# Autodesk Inventor assembly: R2_上昇機構
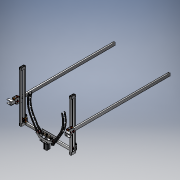
[picture p0: Inventor's stored thumbnail of the model, 180x180]
Saved by Autodesk Inventor 2019.4 (Build 234330000, 330)
## iProperties
Created: 2021-12-04
Part Number: R2_上昇機構
Material: 一般
Document SubType Name: Assembly
Designer: 堀川皓史
Mass: 2467.94 g
Surface Area: 9954.17 cm^2
Volume: 1031.77 cm^3
Density: 2.39196 g/cm^3
Author: 堀川皓史
## Documents named in this file (17)
- C:\Users\堀川皓史\Desktop\ロボ研\NHKフォルダ\2022NHKロボコン\R2_version1\R2_上昇機構.iam
- C:\Users\堀川皓史\Desktop\ロボ研\NHKフォルダ\2022NHKロボコン\R2_version1\上昇機構_内側板.ipt
- C:\Users\堀川皓史\Desktop\ロボ研\NHKフォルダ\2022NHKロボコン\R2_version1\上昇機構_外側板.ipt
- C:\Users\堀川皓史\Desktop\ロボ研\NHKフォルダ\2022NHKロボコン\R2_version1\上昇機構_固定軸ベアリングの.ipt
- C:\Users\堀川皓史\Desktop\ロボ研\NHKフォルダ\2022NHKロボコン\R2_version1\ベアリング_6-19-6.ipt
- C:\Users\堀川皓史\Desktop\ロボ研\NHKフォルダ\2022NHKロボコン\R2_version1\上昇機構_角柱1.ipt
- C:\Users\堀川皓史\Desktop\ロボ研\NHKフォルダ\2022NHKロボコン\R2_version1\上昇機構_固定具1.ipt
- C:\Users\堀川皓史\Desktop\ロボ研\NHKフォルダ\2022NHKロボコン\R2_version1\スペーサ_6.1-7_3Dプリンタ.ipt
- C:\Users\堀川皓史\Desktop\ロボ研\NHKフォルダ\2022NHKロボコン\R2_version1\軸_6-24.ipt
- C:\Users\堀川皓史\Desktop\ロボ研\NHKフォルダ\2022NHKロボコン\R2_version1\上昇機構_角柱3.ipt
- C:\Users\堀川皓史\Desktop\ロボ研\NHKフォルダ\2022NHKロボコン\R2_version1\上昇機構_角柱4.ipt
- C:\Users\堀川皓史\Desktop\ロボ研\NHKフォルダ\2022NHKロボコン\R2_version1\上昇機構_側板1.ipt
- C:\Users\堀川皓史\Desktop\ロボ研\NHKフォルダ\2022NHKロボコン\R2_version1\前後機構_上側板.ipt
- C:\Users\堀川皓史\Desktop\ロボ研\NHKフォルダ\2022NHKロボコン\R2_version1\前後機構_下側板.ipt
- C:\Users\堀川皓史\Desktop\ロボ研\NHKフォルダ\2022NHKロボコン\R2_version1\軸_3.2-8_特殊.ipt
- C:\Users\堀川皓史\Desktop\ロボ研\NHKフォルダ\2022NHKロボコン\R2_version1\ベアリング_3-7-3.ipt
- C:\Users\堀川皓史\Desktop\ロボ研\NHKフォルダ\2022NHKロボコン\R2_version1\R2_ハンド.iam
## Components (97 placed, 16 different names)
1. 上昇機構_内側板:1 — 挿入:57, 挿入:58, メイト:17, 挿入:63, 挿入:66, 挿入:67, 挿入:81, 挿入:82
2. 上昇機構_外側板:1 — 挿入:59, 挿入:60, 挿入:61, 挿入:62, メイト:20, メイト:21, 挿入:72, 挿入:73
3. 上昇機構_固定軸ベアリングの:1 — 挿入:61, 挿入:62, メイト:19
4. 上昇機構_固定軸ベアリングの:2 — 挿入:59, 挿入:60, メイト:18
5. 上昇機構_固定軸ベアリングの:3 — 挿入:57, 挿入:58, メイト:16
6. ベアリング_6-19-6:1 — メイト:16, メイト:17, 正接:4
7. ベアリング_6-19-6:2 — 挿入:70, 正接:5
8. ベアリング_6-19-6:3 — 挿入:71, 正接:2
9. ベアリング_6-19-6:4 — 挿入:65, 正接:3
10. ベアリング_6-19-6:5 — メイト:19, メイト:21
11. ベアリング_6-19-6:6 — メイト:18, メイト:20, 正接:6
12. スペーサ_6.1-7_3Dプリンタ:1 — 挿入:75
13. スペーサ_6.1-7_3Dプリンタ:2 — 挿入:64, 挿入:65
14. スペーサ_6.1-7_3Dプリンタ:3 — 挿入:74
15. スペーサ_6.1-7_3Dプリンタ:4 — 挿入:69, 挿入:71
16. スペーサ_6.1-7_3Dプリンタ:5 — 挿入:76
17. スペーサ_6.1-7_3Dプリンタ:6 — 挿入:68, 挿入:70
18. 軸_6-24:1 — 挿入:67, 挿入:69, 挿入:74
19. 軸_6-24:2 — 挿入:66, 挿入:68, 挿入:73, 挿入:75
20. 軸_6-24:3 — 挿入:63, 挿入:64, 挿入:72, 挿入:76
21. 上昇機構_角柱1:1 — 挿入:31, 挿入:33, 挿入:34, 挿入:35, 正接:2, 正接:3, 正接:4, 正接:5, 正接:6
22. 上昇機構_固定具1:1 — 挿入:31, 挿入:35
23. 上昇機構_固定具1:2 — 挿入:33, 挿入:34, フラッシュ:1
24. 上昇機構_内側板:2 — 挿入:103, 挿入:104
25. 上昇機構_外側板:2
26. 上昇機構_固定軸ベアリングの:4
27. 上昇機構_固定軸ベアリングの:5
28. 上昇機構_固定軸ベアリングの:6
29. ベアリング_6-19-6:7 — 正接:12
30. ベアリング_6-19-6:8 — 正接:7
31. ベアリング_6-19-6:9 — 正接:8
32. ベアリング_6-19-6:10 — 正接:11
33. ベアリング_6-19-6:11 — 正接:10
34. ベアリング_6-19-6:12 — 正接:9
35. スペーサ_6.1-7_3Dプリンタ:7
36. スペーサ_6.1-7_3Dプリンタ:8
37. スペーサ_6.1-7_3Dプリンタ:9
38. スペーサ_6.1-7_3Dプリンタ:10
39. スペーサ_6.1-7_3Dプリンタ:11
40. スペーサ_6.1-7_3Dプリンタ:12
41. 軸_6-24:4
42. 軸_6-24:5
43. 軸_6-24:6
44. 上昇機構_角柱1:2 — 正接:7, 正接:8, 正接:9, 正接:10, 正接:11, 正接:12
45. 上昇機構_固定具1:3 — フラッシュ:1
46. 上昇機構_固定具1:4
47. 上昇機構_角柱3:1 — 挿入:81, 挿入:82, 挿入:83, 挿入:84, 挿入:85, 挿入:86, 挿入:87, 挿入:88
48. 上昇機構_角柱4:1 — 挿入:89, 挿入:90, 挿入:91, 挿入:92, 正接:15, 正接:16, 正接:17, 正接:18, 正接:19, 正接:20
49. 上昇機構_側板1:1 — 挿入:83, 挿入:84, 挿入:92
50. 上昇機構_側板1:2 — 挿入:85, 挿入:86, 挿入:90
51. 上昇機構_側板1:3 — 挿入:87, 挿入:91
52. 上昇機構_側板1:4 — 挿入:88, 挿入:89
53. 上昇機構_角柱3:2 — 挿入:103, 挿入:104
54. 上昇機構_角柱4:2 — 正接:21, 正接:22, 正接:23, 正接:24
55. 上昇機構_側板1:5
56. 上昇機構_側板1:6
57. 上昇機構_側板1:7
58. 上昇機構_側板1:8
59. 前後機構_上側板:1 — 挿入:109, 挿入:110, 挿入:114, 挿入:131, 挿入:132, メイト:28, 挿入:133, 挿入:134, メイト:29, 挿入:143, 挿入:144
60. 前後機構_上側板:2 — 挿入:105, 挿入:106, 挿入:115, 挿入:137, 挿入:138, 挿入:139, 挿入:140, メイト:32, メイト:33, 挿入:145, 挿入:146
61. 前後機構_下側板:1 — 挿入:107, 挿入:108, 挿入:116, 挿入:141, 挿入:142, メイト:31
62. 前後機構_下側板:2 — 挿入:111, 挿入:112, 挿入:113, 挿入:135, 挿入:136, メイト:30
63. 軸_6-24:7 — 挿入:105, 挿入:107, 挿入:125, 挿入:126
64. 軸_6-24:8 — 挿入:106, 挿入:108, 挿入:123, 挿入:124
65. 軸_6-24:9 — 挿入:109, 挿入:111, 挿入:128, 挿入:130
66. 軸_6-24:10 — 挿入:110, 挿入:112, 挿入:127, 挿入:129
67. 軸_3.2-8_特殊:1 — 挿入:113, 挿入:118
68. 軸_3.2-8_特殊:2 — 挿入:114
69. 軸_3.2-8_特殊:3 — 挿入:115
70. 軸_3.2-8_特殊:4 — 挿入:116, 挿入:117
71. ベアリング_3-7-3:1 — 挿入:117, 正接:21
72. ベアリング_3-7-3:2 — 挿入:118
73. ベアリング_6-19-6:13 — 正接:23
74. スペーサ_6.1-7_3Dプリンタ:13 — 挿入:123
75. スペーサ_6.1-7_3Dプリンタ:14 — 挿入:124
76. ベアリング_6-19-6:14 — 正接:24
77. スペーサ_6.1-7_3Dプリンタ:15 — 挿入:125
78. スペーサ_6.1-7_3Dプリンタ:16 — 挿入:126
79. ベアリング_6-19-6:15 — 正接:15
80. スペーサ_6.1-7_3Dプリンタ:17 — 挿入:128
81. スペーサ_6.1-7_3Dプリンタ:18 — 挿入:130
82. ベアリング_6-19-6:16 — 正接:20
83. スペーサ_6.1-7_3Dプリンタ:19 — 挿入:127
84. スペーサ_6.1-7_3Dプリンタ:20 — 挿入:129
85. 上昇機構_固定軸ベアリングの:7 — 挿入:133, 挿入:134
86. ベアリング_6-19-6:17 — メイト:29, 正接:19
87. 上昇機構_固定軸ベアリングの:8 — 挿入:131, 挿入:132
88. ベアリング_6-19-6:18 — メイト:28, 正接:16, 正接:18
89. 上昇機構_固定軸ベアリングの:9 — 挿入:137, 挿入:138
90. ベアリング_6-19-6:19 — メイト:32, 正接:22
91. 上昇機構_固定軸ベアリングの:10 — 挿入:139, 挿入:140
92. ベアリング_6-19-6:20 — メイト:33
93. 上昇機構_固定軸ベアリングの:11 — 挿入:141, 挿入:142
94. ベアリング_6-19-6:21 — メイト:31
95. 上昇機構_固定軸ベアリングの:12 — 挿入:135, 挿入:136
96. ベアリング_6-19-6:22 — メイト:30, 正接:17
97. R2_ハンド:1 [sub-assembly] — 挿入:143, 挿入:144, 挿入:145, 挿入:146
## Relationships (161: Insert 115, Mate 24, Tangent 21, Flush 1)
- 挿入:31 [Insert]: 上昇機構_角柱1:1 ↔ 上昇機構_固定具1:1
- 挿入:33 [Insert]: 上昇機構_角柱1:1 ↔ 上昇機構_固定具1:2
- 挿入:34 [Insert]: 上昇機構_角柱1:1 ↔ 上昇機構_固定具1:2
- 挿入:35 [Insert]: 上昇機構_角柱1:1 ↔ 上昇機構_固定具1:1
- [Insert]: 上昇機構_内側板:2 ↔ 上昇機構_固定軸ベアリングの:6
- [Insert]: 上昇機構_内側板:2 ↔ 上昇機構_固定軸ベアリングの:6
- [Insert]: 上昇機構_外側板:2 ↔ 上昇機構_固定軸ベアリングの:5
- [Insert]: 上昇機構_外側板:2 ↔ 上昇機構_固定軸ベアリングの:5
- [Insert]: 上昇機構_外側板:2 ↔ 上昇機構_固定軸ベアリングの:4
- [Insert]: 上昇機構_外側板:2 ↔ 上昇機構_固定軸ベアリングの:4
- [Mate]: 上昇機構_固定軸ベアリングの:6 ↔ ベアリング_6-19-6:7
- [Mate] (0.1 mm): 上昇機構_内側板:2 ↔ ベアリング_6-19-6:7
- [Mate]: 上昇機構_固定軸ベアリングの:5 ↔ ベアリング_6-19-6:12
- [Mate]: 上昇機構_固定軸ベアリングの:4 ↔ ベアリング_6-19-6:11
- [Mate] (0.1 mm): 上昇機構_外側板:2 ↔ ベアリング_6-19-6:12
- [Mate] (0.1 mm): 上昇機構_外側板:2 ↔ ベアリング_6-19-6:11
- [Insert]: 上昇機構_内側板:2 ↔ 軸_6-24:4
- [Insert]: 上昇機構_内側板:2 ↔ 軸_6-24:5
- [Insert]: 上昇機構_内側板:2 ↔ 軸_6-24:6
- [Insert]: 上昇機構_外側板:2 ↔ 軸_6-24:6
- [Insert]: 上昇機構_外側板:2 ↔ 軸_6-24:5
- [Insert]: 上昇機構_外側板:2 ↔ 軸_6-24:4
- [Insert]: ベアリング_6-19-6:8 ↔ スペーサ_6.1-7_3Dプリンタ:7
- [Insert]: スペーサ_6.1-7_3Dプリンタ:7 ↔ 軸_6-24:5
- [Insert]: スペーサ_6.1-7_3Dプリンタ:12 ↔ 軸_6-24:5
- [Insert]: スペーサ_6.1-7_3Dプリンタ:10 ↔ 軸_6-24:4
- [Insert]: スペーサ_6.1-7_3Dプリンタ:11 ↔ 軸_6-24:4
- [Insert]: スペーサ_6.1-7_3Dプリンタ:9 ↔ 軸_6-24:6
- [Insert]: スペーサ_6.1-7_3Dプリンタ:8 ↔ 軸_6-24:6
- [Insert]: ベアリング_6-19-6:10 ↔ スペーサ_6.1-7_3Dプリンタ:8
- [Insert]: ベアリング_6-19-6:9 ↔ スペーサ_6.1-7_3Dプリンタ:10
- 挿入:57 [Insert]: 上昇機構_内側板:1 ↔ 上昇機構_固定軸ベアリングの:3
- 挿入:58 [Insert]: 上昇機構_内側板:1 ↔ 上昇機構_固定軸ベアリングの:3
- メイト:16 [Mate]: 上昇機構_固定軸ベアリングの:3 ↔ ベアリング_6-19-6:1
- メイト:17 [Mate] (0.1 mm): 上昇機構_内側板:1 ↔ ベアリング_6-19-6:1
- 挿入:59 [Insert]: 上昇機構_外側板:1 ↔ 上昇機構_固定軸ベアリングの:2
- 挿入:60 [Insert]: 上昇機構_外側板:1 ↔ 上昇機構_固定軸ベアリングの:2
- 挿入:61 [Insert]: 上昇機構_外側板:1 ↔ 上昇機構_固定軸ベアリングの:1
- 挿入:62 [Insert]: 上昇機構_外側板:1 ↔ 上昇機構_固定軸ベアリングの:1
- メイト:18 [Mate]: 上昇機構_固定軸ベアリングの:2 ↔ ベアリング_6-19-6:6
- メイト:19 [Mate]: 上昇機構_固定軸ベアリングの:1 ↔ ベアリング_6-19-6:5
- メイト:20 [Mate]: 上昇機構_外側板:1 ↔ ベアリング_6-19-6:6
- メイト:21 [Mate] (0.1 mm): 上昇機構_外側板:1 ↔ ベアリング_6-19-6:5
- 挿入:63 [Insert]: 上昇機構_内側板:1 ↔ 軸_6-24:3
- 挿入:64 [Insert]: スペーサ_6.1-7_3Dプリンタ:2 ↔ 軸_6-24:3
- 挿入:65 [Insert]: ベアリング_6-19-6:4 ↔ スペーサ_6.1-7_3Dプリンタ:2
- 挿入:66 [Insert]: 上昇機構_内側板:1 ↔ 軸_6-24:2
- 挿入:67 [Insert]: 上昇機構_内側板:1 ↔ 軸_6-24:1
- 挿入:68 [Insert]: スペーサ_6.1-7_3Dプリンタ:6 ↔ 軸_6-24:2
- 挿入:69 [Insert]: スペーサ_6.1-7_3Dプリンタ:4 ↔ 軸_6-24:1
- 挿入:70 [Insert]: ベアリング_6-19-6:2 ↔ スペーサ_6.1-7_3Dプリンタ:6
- 挿入:71 [Insert]: ベアリング_6-19-6:3 ↔ スペーサ_6.1-7_3Dプリンタ:4
- 挿入:72 [Insert]: 上昇機構_外側板:1 ↔ 軸_6-24:3
- 挿入:73 [Insert]: 上昇機構_外側板:1 ↔ 軸_6-24:2
- 挿入:74 [Insert]: スペーサ_6.1-7_3Dプリンタ:3 ↔ 軸_6-24:1
- 挿入:75 [Insert]: スペーサ_6.1-7_3Dプリンタ:1 ↔ 軸_6-24:2
- 挿入:76 [Insert]: スペーサ_6.1-7_3Dプリンタ:5 ↔ 軸_6-24:3
- 正接:2 [Tangent]: ベアリング_6-19-6:3 ↔ 上昇機構_角柱1:1
- 正接:3 [Tangent]: ベアリング_6-19-6:4 ↔ 上昇機構_角柱1:1
- 正接:4 [Tangent]: ベアリング_6-19-6:1 ↔ 上昇機構_角柱1:1
- 正接:5 [Tangent]: ベアリング_6-19-6:2 ↔ 上昇機構_角柱1:1
- 正接:6 [Tangent]: ベアリング_6-19-6:6 ↔ 上昇機構_角柱1:1
- [Insert]: 上昇機構_角柱1:2 ↔ 上昇機構_固定具1:3
- [Insert]: 上昇機構_角柱1:2 ↔ 上昇機構_固定具1:4
- [Insert]: 上昇機構_角柱1:2 ↔ 上昇機構_固定具1:4
- [Insert]: 上昇機構_角柱1:2 ↔ 上昇機構_固定具1:3
- 挿入:81 [Insert]: 上昇機構_内側板:1 ↔ 上昇機構_角柱3:1
- 挿入:82 [Insert]: 上昇機構_内側板:1 ↔ 上昇機構_角柱3:1
- 挿入:83 [Insert]: 上昇機構_角柱3:1 ↔ 上昇機構_側板1:1
- 挿入:84 [Insert]: 上昇機構_角柱3:1 ↔ 上昇機構_側板1:1
- 挿入:85 [Insert]: 上昇機構_角柱3:1 ↔ 上昇機構_側板1:2
- 挿入:86 [Insert]: 上昇機構_角柱3:1 ↔ 上昇機構_側板1:2
- 挿入:87 [Insert]: 上昇機構_角柱3:1 ↔ 上昇機構_側板1:3
- 挿入:88 [Insert]: 上昇機構_角柱3:1 ↔ 上昇機構_側板1:4
- 挿入:89 [Insert]: 上昇機構_角柱4:1 ↔ 上昇機構_側板1:4
- 挿入:90 [Insert]: 上昇機構_角柱4:1 ↔ 上昇機構_側板1:2
- 挿入:91 [Insert]: 上昇機構_角柱4:1 ↔ 上昇機構_側板1:3
- 挿入:92 [Insert]: 上昇機構_角柱4:1 ↔ 上昇機構_側板1:1
- 正接:7 [Tangent]: ベアリング_6-19-6:8 ↔ 上昇機構_角柱1:2
- 正接:8 [Tangent]: ベアリング_6-19-6:9 ↔ 上昇機構_角柱1:2
- 正接:9 [Tangent]: ベアリング_6-19-6:12 ↔ 上昇機構_角柱1:2
- 正接:10 [Tangent]: ベアリング_6-19-6:11 ↔ 上昇機構_角柱1:2
- 正接:11 [Tangent]: ベアリング_6-19-6:10 ↔ 上昇機構_角柱1:2
- 正接:12 [Tangent]: ベアリング_6-19-6:7 ↔ 上昇機構_角柱1:2
- [Insert]: 上昇機構_角柱3:2 ↔ 上昇機構_側板1:5
- [Insert]: 上昇機構_角柱3:2 ↔ 上昇機構_側板1:5
- [Insert]: 上昇機構_角柱3:2 ↔ 上昇機構_側板1:6
- [Insert]: 上昇機構_角柱3:2 ↔ 上昇機構_側板1:6
- [Insert]: 上昇機構_角柱3:2 ↔ 上昇機構_側板1:7
- [Insert]: 上昇機構_角柱3:2 ↔ 上昇機構_側板1:8
- [Insert]: 上昇機構_角柱4:2 ↔ 上昇機構_側板1:8
- [Insert]: 上昇機構_角柱4:2 ↔ 上昇機構_側板1:6
- [Insert]: 上昇機構_角柱4:2 ↔ 上昇機構_側板1:7
- [Insert]: 上昇機構_角柱4:2 ↔ 上昇機構_側板1:5
- 挿入:103 [Insert]: 上昇機構_内側板:2 ↔ 上昇機構_角柱3:2
- 挿入:104 [Insert]: 上昇機構_内側板:2 ↔ 上昇機構_角柱3:2
- 挿入:105 [Insert]: 前後機構_上側板:2 ↔ 軸_6-24:7
- 挿入:106 [Insert]: 前後機構_上側板:2 ↔ 軸_6-24:8
- 挿入:107 [Insert]: 前後機構_下側板:1 ↔ 軸_6-24:7
- 挿入:108 [Insert]: 前後機構_下側板:1 ↔ 軸_6-24:8
- 挿入:109 [Insert]: 前後機構_上側板:1 ↔ 軸_6-24:9
- 挿入:110 [Insert]: 前後機構_上側板:1 ↔ 軸_6-24:10
- 挿入:111 [Insert]: 前後機構_下側板:2 ↔ 軸_6-24:9
- 挿入:112 [Insert]: 前後機構_下側板:2 ↔ 軸_6-24:10
- 挿入:113 [Insert]: 前後機構_下側板:2 ↔ 軸_3.2-8_特殊:1
- 挿入:114 [Insert]: 前後機構_上側板:1 ↔ 軸_3.2-8_特殊:2
- 挿入:115 [Insert]: 前後機構_上側板:2 ↔ 軸_3.2-8_特殊:3
- 挿入:116 [Insert]: 前後機構_下側板:1 ↔ 軸_3.2-8_特殊:4
- 挿入:117 [Insert]: 軸_3.2-8_特殊:4 ↔ ベアリング_3-7-3:1
- 挿入:118 [Insert]: 軸_3.2-8_特殊:1 ↔ ベアリング_3-7-3:2
- [Insert]: ベアリング_6-19-6:13 ↔ スペーサ_6.1-7_3Dプリンタ:13
- [Insert]: ベアリング_6-19-6:14 ↔ スペーサ_6.1-7_3Dプリンタ:15
- [Insert]: ベアリング_6-19-6:15 ↔ スペーサ_6.1-7_3Dプリンタ:17
- [Insert]: ベアリング_6-19-6:16 ↔ スペーサ_6.1-7_3Dプリンタ:19
- 挿入:123 [Insert]: 軸_6-24:8 ↔ スペーサ_6.1-7_3Dプリンタ:13
- 挿入:124 [Insert]: 軸_6-24:8 ↔ スペーサ_6.1-7_3Dプリンタ:14
- 挿入:125 [Insert]: 軸_6-24:7 ↔ スペーサ_6.1-7_3Dプリンタ:15
- 挿入:126 [Insert]: 軸_6-24:7 ↔ スペーサ_6.1-7_3Dプリンタ:16
- 挿入:127 [Insert]: 軸_6-24:10 ↔ スペーサ_6.1-7_3Dプリンタ:19
- 挿入:128 [Insert]: 軸_6-24:9 ↔ スペーサ_6.1-7_3Dプリンタ:17
- 挿入:129 [Insert]: 軸_6-24:10 ↔ スペーサ_6.1-7_3Dプリンタ:20
- 挿入:130 [Insert]: 軸_6-24:9 ↔ スペーサ_6.1-7_3Dプリンタ:18
- [Mate]: 上昇機構_固定軸ベアリングの:7 ↔ ベアリング_6-19-6:17
- [Mate]: 上昇機構_固定軸ベアリングの:8 ↔ ベアリング_6-19-6:18
- [Mate]: 上昇機構_固定軸ベアリングの:9 ↔ ベアリング_6-19-6:19
- [Mate]: 上昇機構_固定軸ベアリングの:10 ↔ ベアリング_6-19-6:20
- [Mate]: 上昇機構_固定軸ベアリングの:11 ↔ ベアリング_6-19-6:21
- [Mate]: 上昇機構_固定軸ベアリングの:12 ↔ ベアリング_6-19-6:22
- 挿入:131 [Insert]: 前後機構_上側板:1 ↔ 上昇機構_固定軸ベアリングの:8
- 挿入:132 [Insert]: 前後機構_上側板:1 ↔ 上昇機構_固定軸ベアリングの:8
- メイト:28 [Mate] (0.1 mm): 前後機構_上側板:1 ↔ ベアリング_6-19-6:18
- 挿入:133 [Insert]: 前後機構_上側板:1 ↔ 上昇機構_固定軸ベアリングの:7
- 挿入:134 [Insert]: 前後機構_上側板:1 ↔ 上昇機構_固定軸ベアリングの:7
- 挿入:135 [Insert]: 前後機構_下側板:2 ↔ 上昇機構_固定軸ベアリングの:12
- 挿入:136 [Insert]: 前後機構_下側板:2 ↔ 上昇機構_固定軸ベアリングの:12
- メイト:29 [Mate] (0.1 mm): 前後機構_上側板:1 ↔ ベアリング_6-19-6:17
- メイト:30 [Mate] (0.1 mm): 前後機構_下側板:2 ↔ ベアリング_6-19-6:22
- 挿入:137 [Insert]: 前後機構_上側板:2 ↔ 上昇機構_固定軸ベアリングの:9
- 挿入:138 [Insert]: 前後機構_上側板:2 ↔ 上昇機構_固定軸ベアリングの:9
- 挿入:139 [Insert]: 前後機構_上側板:2 ↔ 上昇機構_固定軸ベアリングの:10
- 挿入:140 [Insert]: 前後機構_上側板:2 ↔ 上昇機構_固定軸ベアリングの:10
- 挿入:141 [Insert]: 前後機構_下側板:1 ↔ 上昇機構_固定軸ベアリングの:11
- 挿入:142 [Insert]: 前後機構_下側板:1 ↔ 上昇機構_固定軸ベアリングの:11
- メイト:31 [Mate] (0.1 mm): 前後機構_下側板:1 ↔ ベアリング_6-19-6:21
- メイト:32 [Mate] (0.1 mm): 前後機構_上側板:2 ↔ ベアリング_6-19-6:19
- メイト:33 [Mate] (0.1 mm): 前後機構_上側板:2 ↔ ベアリング_6-19-6:20
- フラッシュ:1 [Flush]: 上昇機構_固定具1:2 ↔ 上昇機構_固定具1:3
- 正接:15 [Tangent]: 上昇機構_角柱4:1 ↔ ベアリング_6-19-6:15
- 正接:16 [Tangent]: 上昇機構_角柱4:1 ↔ ベアリング_6-19-6:18
- 正接:17 [Tangent]: 上昇機構_角柱4:1 ↔ ベアリング_6-19-6:22
- 正接:18 [Tangent]: 上昇機構_角柱4:1 ↔ ベアリング_6-19-6:18
- 正接:19 [Tangent]: 上昇機構_角柱4:1 ↔ ベアリング_6-19-6:17
- 正接:20 [Tangent]: 上昇機構_角柱4:1 ↔ ベアリング_6-19-6:16
- 正接:21 [Tangent]: 上昇機構_角柱4:2 ↔ ベアリング_3-7-3:1
- 正接:22 [Tangent]: 上昇機構_角柱4:2 ↔ ベアリング_6-19-6:19
- 正接:23 [Tangent]: 上昇機構_角柱4:2 ↔ ベアリング_6-19-6:13
- 正接:24 [Tangent]: 上昇機構_角柱4:2 ↔ ベアリング_6-19-6:14
- 挿入:143 [Insert]: 前後機構_上側板:1 ↔ R2_ハンド:1
- 挿入:144 [Insert]: 前後機構_上側板:1 ↔ R2_ハンド:1
- 挿入:145 [Insert]: 前後機構_上側板:2 ↔ R2_ハンド:1
- 挿入:146 [Insert]: 前後機構_上側板:2 ↔ R2_ハンド:1
## Named parameters: d65_d52 = 0 mm, d66_d44 = 0 mm, d67_d45 = 0 mm, d68_d46 = 0 mm, d69_d47 = 0 mm, d70_d48 = 0 mm, d71_d49 = 0 mm, d72_d50 = 0 mm, d73_d51 = 0 mm, d74_d18 = 0.1 mm, d75_d19 = 0.1 mm, d76_d5 = 0 mm, d77_d6 = 0 mm, d78_d7 = 0 mm, d79_d8 = 0 mm, d80_d9 = 0 mm, d81_d10 = 0 mm, d82_d11 = 0 mm, d83_d12 = 0.1 mm, d84_d13 = 0 mm, d85_d14 = 0 mm, d86_d38 = 0 mm, d87_d39 = 0 mm, d88_d40 = 0 mm, d89_d41 = 0 mm, d90_d42 = 0 mm, d91_d43 = 0 mm, d124_d63 = 0 mm, d125_d64 = 0 mm, d126_d53 = 0 mm, d127_d55 = 0 mm, d163_d136 = 0 mm, d164_d137 = 0 mm, d165_d138 = 0 mm, d166_d139 = 0 mm, d167_d140 = 0 mm, d168_d141 = 0 mm, d169_d142 = 0 mm, d170_d143 = 0 mm, d171_d144 = 0 mm, d172_d145 = 0 mm, d189_d73_d51 = 0 mm, d190_d73_d51 = 0 mm, d191_d73_d51 = 0 mm, d192_d73_d51 = 0 mm, d201_d100 = 0 mm, d202_d100 = 0 mm, d203_d100 = 0 mm, d204_d100 = 0 mm, d205_d100 = 0 mm, d206_d100 = 0 mm
